# Autodesk Inventor assembly: X rail T + dual mount
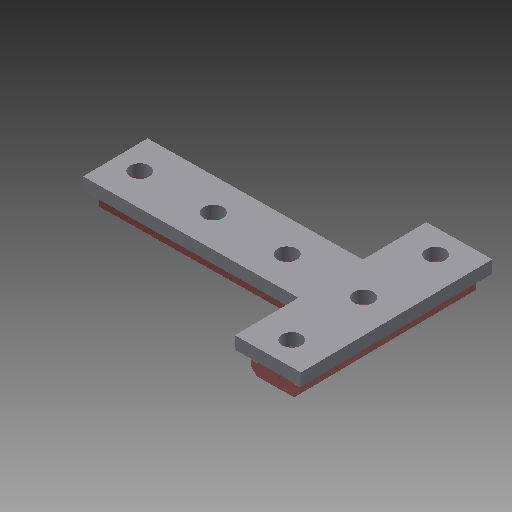
[picture p0: Inventor's stored thumbnail of the model, 512x512]
Saved by Autodesk Inventor 2018 (Build 220112000, 112)
## iProperties
Created: 2017-11-10
Part Number: X rail T + dual mount
Document SubType Name: Assembly
Designer: ball
Author: ball
## Documents named in this file (3)
- C:\FTC\2017Robot\X rail T + dual mount.iam
- C:\FTC\Actobotics\585 parts\585718.ipt
- C:\FTC\Actobotics\585 parts\585075.ipt
## Components (3 placed, 2 different names)
1. 585718:1
2. 585075:1 — Mate:4, Mate:5, Mate:6
3. 585718:2 — Mate:4, Mate:5, Mate:6
## Relationships (6: Mate 6)
- [Mate]: 585718:1 ↔ 585075:1
- [Mate]: 585718:1 ↔ 585075:1
- [Mate]: 585718:1 ↔ 585075:1
- Mate:4: 585075:1 ↔ 585718:2
- Mate:5: 585075:1 ↔ 585718:2
- Mate:6: 585075:1 ↔ 585718:2
